# Autodesk Inventor assembly: noga podest duzy
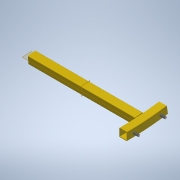
[picture p0: Inventor's stored thumbnail of the model, 180x180]
Saved by Autodesk Inventor 2021 (Build 250183000, 183)
## iProperties
Created: 2024-04-18
Part Number: noga podest duzy
Document SubType Name: Assembly
Designer: Michal
Author: Michal
## Documents named in this file (4)
- C:\Users\Michal\Documents\GitHub\PNW_PhotoBoothFrame_3D\noga podest duzy.iam
- C:\Users\Michal\Documents\GitHub\PNW_PhotoBoothFrame_3D\podest duzy profil 7.ipt
- C:\Users\Michal\Documents\GitHub\PNW_PhotoBoothFrame_3D\M8x50.ipt
- C:\Users\Michal\Documents\GitHub\PNW_PhotoBoothFrame_3D\podest duzy profil 8.ipt
## Components (4 placed, 3 different names)
1. podest duzy profil 7:1 — Mate:11, Mate:12, Mate:13, Flush:2, Mate:14
2. M8x50:1 — Flush:1, Mate:12, Mate:13
3. M8x50:2 — Flush:1, Mate:11
4. podest duzy profil 8:1 — Flush:2, Mate:14
## Relationships (6: Mate 4, Flush 2)
- Flush:1: M8x50:1 ↔ M8x50:2
- Mate:11: podest duzy profil 7:1 ↔ M8x50:2
- Mate:12: podest duzy profil 7:1 ↔ M8x50:1
- Mate:13: podest duzy profil 7:1 ↔ M8x50:1
- Flush:2: podest duzy profil 7:1 ↔ podest duzy profil 8:1
- Mate:14: podest duzy profil 7:1 ↔ podest duzy profil 8:1
